# Autodesk Inventor assembly: BoltWasher4x10
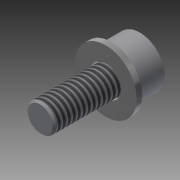
[picture p0: Inventor's stored thumbnail of the model, 180x180]
Saved by Autodesk Inventor 2015 SP1 (Build 190203100, 203)
## iProperties
Category: Hardware
Created: 2015-01-27
Part Number: BoltWasher4x10
Document SubType Name: Assembly
Designer: Jack
Vendor: Misumi
Author: Jack
Title: Bolt + Washer 3x24
## Documents named in this file (3)
- C:\Users\Jack\ownCloud\Projects\CrossBot\InventorModel\Hardware\BoltWashers\BoltWasher4\BoltWasher4x10.iam
- C:\Users\Jack\ownCloud\Projects\CrossBot\InventorModel\Hardware\Wahsers\M4Washer.ipt
- C:\Users\Jack\ownCloud\Projects\CrossBot\InventorModel\Hardware\Bolts\SHCS\SHCS4\SHCS4x10.ipt
## Components (2 placed, 2 different names)
1. M4Washer:1 — Mate:1, Mate:2
2. SHCS4x10:1 — Mate:1, Mate:2
## Relationships (2: Mate 2)
- Mate:1: M4Washer:1 ↔ SHCS4x10:1
- Mate:2: M4Washer:1 ↔ SHCS4x10:1
